# Autodesk Inventor assembly: Baugruppe1
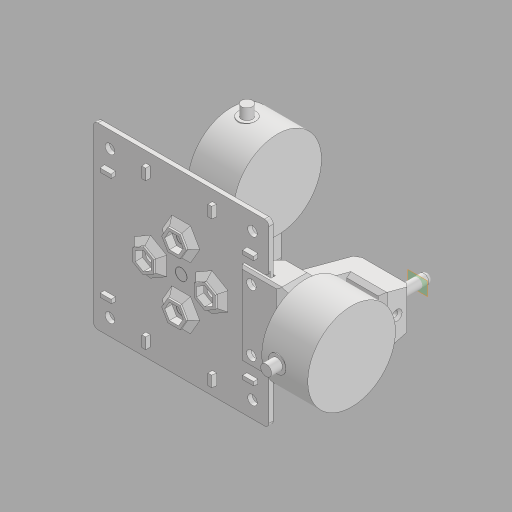
[picture p0: Inventor's stored thumbnail of the model, 512x512]
Saved by Autodesk Inventor 2023 (Build 270158000, 158)
## iProperties
Created: 2024-12-10
Part Number: Baugruppe1
Document SubType Name: Assembly
Designer: Nils Bade
Author: Nils Bade
## Documents named in this file (6)
- C:\Users\Nils Bade\Documents\Projektarbeit_Bade\GIT\Masterarbeit-Inventor\Baugruppe1.iam
- MessuhrHalterAssembly.iam
- C:\Users\Nils Bade\Documents\Projektarbeit_Bade\GIT\Masterarbeit-Inventor\RatRig_modified\ProbeHead\ProbeAntennas\Vermessungsbauteile\MessuhrHalter-BasePlate.ipt
- C:\Users\Nils Bade\Documents\Projektarbeit_Bade\GIT\Masterarbeit-Inventor\RatRig_modified\ProbeHead\ProbeAntennas\Vermessungsbauteile\MessuhrXYKlemme.ipt
- C:\Users\Nils Bade\Documents\Projektarbeit_Bade\GIT\Masterarbeit-Inventor\RatRig_modified\ProbeHead\ProbeAntennas\Vermessungsbauteile\MessuhrZKlemme.ipt
- C:\Users\Nils Bade\Documents\Projektarbeit_Bade\GIT\Masterarbeit-Inventor\RatRig_modified\ProbeHead\ProbeAntennas\Vermessungsbauteile\Messuhr-Dummy.ipt
## Components (5 placed, 4 different names)
1. MessuhrHalter-BasePlate:1 — Passend:1, Passend:2, Passend:3, Passend:4, Passend:5, Passend:6
2. MessuhrXYKlemme:1 — Passend:1, Passend:2, Passend:6, Tangential:2, Passend:8
3. MessuhrZKlemme:1 — Passend:3, Passend:4, Passend:5, Passend:7, Tangential:1
4. Messuhr-Dummy:1 — Tangential:2, Passend:8
5. Messuhr-Dummy:2 — Passend:7, Tangential:1
## Relationships (10: Mate 8, Tangent 2)
- Passend:1 [Mate]: MessuhrHalter-BasePlate:1 ↔ MessuhrXYKlemme:1
- Passend:2 [Mate]: MessuhrHalter-BasePlate:1 ↔ MessuhrXYKlemme:1
- Passend:3 [Mate]: MessuhrHalter-BasePlate:1 ↔ MessuhrZKlemme:1
- Passend:4 [Mate]: MessuhrHalter-BasePlate:1 ↔ MessuhrZKlemme:1
- Passend:5 [Mate]: MessuhrHalter-BasePlate:1 ↔ MessuhrZKlemme:1
- Passend:6 [Mate]: MessuhrHalter-BasePlate:1 ↔ MessuhrXYKlemme:1
- Passend:7 [Mate]: MessuhrZKlemme:1 ↔ Messuhr-Dummy:2
- Tangential:1: MessuhrZKlemme:1 ↔ Messuhr-Dummy:2
- Tangential:2: MessuhrXYKlemme:1 ↔ Messuhr-Dummy:1
- Passend:8 [Mate]: MessuhrXYKlemme:1 ↔ Messuhr-Dummy:1
